# Autodesk Inventor assembly: winch MK3
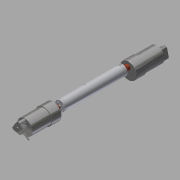
[picture p0: Inventor's stored thumbnail of the model, 180x180]
Saved by Autodesk Inventor 2013 (Build 170138000, 138)
## iProperties
Created: 2013-12-16
Part Number: winch MK3
Document SubType Name: Assembly
Designer: kahohbein
Author: kahohbein
## Documents named in this file (4)
- C:\Users\kahohbein\Documents\GitHub\2013-2014_BlockParty\CAD\Lift\MK3\winch MK3.iam
- C:\Users\kahohbein\Documents\GitHub\2013-2014_BlockParty\CAD\COTSParts\Structural\PVC Spacer 500 Sched 40.ipt
- C:\Users\kahohbein\Documents\GitHub\2013-2014_BlockParty\CAD\COTSParts\Tetrix\Tetrix motor.ipt
- C:\Users\kahohbein\Documents\GitHub\2013-2014_BlockParty\CAD\COTSParts\Tetrix\Tetrix Hub - axle.ipt
## Components (5 placed, 3 different names)
1. PVC Spacer 500 Sched 40:1 — Mate:7, Mate:28, Mate:29, Mate:30, Mate:31
2. Tetrix motor:1
3. Tetrix motor:2 — Mate:7
4. Tetrix Hub - axle:1 — Mate:28, Mate:31
5. Tetrix Hub - axle:2 — Mate:29, Mate:30
## Relationships (5: Mate 5)
- Mate:7: PVC Spacer 500 Sched 40:1 ↔ Tetrix motor:2
- Mate:28: PVC Spacer 500 Sched 40:1 ↔ Tetrix Hub - axle:1
- Mate:29: PVC Spacer 500 Sched 40:1 ↔ Tetrix Hub - axle:2
- Mate:30: PVC Spacer 500 Sched 40:1 ↔ Tetrix Hub - axle:2
- Mate:31: PVC Spacer 500 Sched 40:1 ↔ Tetrix Hub - axle:1
